# Autodesk Inventor assembly: KickerPCB_Unit
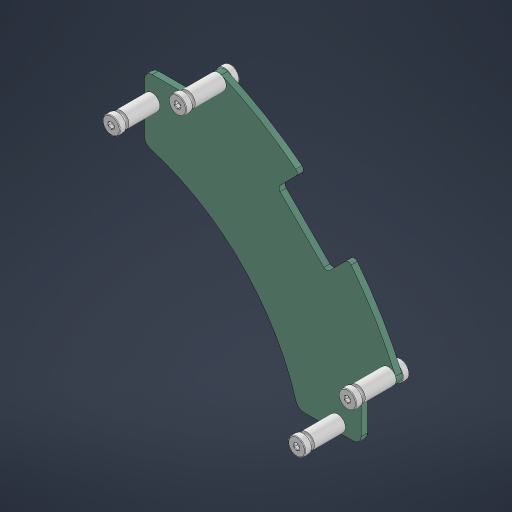
[picture p0: Inventor's stored thumbnail of the model, 512x512]
Saved by Autodesk Inventor 2024.2 (Build 282272000, 272)
## iProperties
Created: 2024-01-10
Part Number: KickerPCB_Unit
Document SubType Name: Assembly
Designer: Hanaoka
Author: Hanaoka
## Documents named in this file (4)
- G:\共有ドライブ\reRo\05_個人\hanaoka\inventor\PCBs\KickerPCB_Unit.iam
- G:\共有ドライブ\reRo\05_個人\hanaoka\inventor\PCBs\MotorDriver_PCB.ipt
- G:\共有ドライブ\reRo\05_個人\hanaoka\inventor\Spacer\Spacer_M2x8.ipt
- G:\共有ドライブ\reRo\05_個人\hanaoka\inventor\Screw\M2x4\M2x4.ipt
## Components (13 placed, 3 different names)
1. MotorDriver_PCB:1 — 挿入:1, 挿入:2, 挿入:3, 挿入:4, 挿入:9, 挿入:10, 挿入:11, 挿入:12
2. Spacer_M2x8:1 — 挿入:4, 挿入:8
3. Spacer_M2x8:2 — 挿入:2, 挿入:6
4. Spacer_M2x8:3 — 挿入:3, 挿入:7
5. Spacer_M2x8:4 — 挿入:1, 挿入:5
6. M2x4:1 — 挿入:5
7. M2x4:2 — 挿入:7
8. M2x4:3 — 挿入:6
9. M2x4:4 — 挿入:8
10. M2x4:5 — 挿入:9
11. M2x4:6 — 挿入:10
12. M2x4:7 — 挿入:11
13. M2x4:8 — 挿入:12
## Relationships (12: Insert 12)
- 挿入:1 [Insert]: MotorDriver_PCB:1 ↔ Spacer_M2x8:4
- 挿入:2 [Insert]: MotorDriver_PCB:1 ↔ Spacer_M2x8:2
- 挿入:3 [Insert]: MotorDriver_PCB:1 ↔ Spacer_M2x8:3
- 挿入:4 [Insert]: MotorDriver_PCB:1 ↔ Spacer_M2x8:1
- 挿入:5 [Insert] (1 mm): Spacer_M2x8:4 ↔ M2x4:1
- 挿入:6 [Insert] (1 mm): Spacer_M2x8:2 ↔ M2x4:3
- 挿入:7 [Insert] (1 mm): Spacer_M2x8:3 ↔ M2x4:2
- 挿入:8 [Insert] (1 mm): Spacer_M2x8:1 ↔ M2x4:4
- 挿入:9 [Insert]: MotorDriver_PCB:1 ↔ M2x4:5
- 挿入:10 [Insert]: MotorDriver_PCB:1 ↔ M2x4:6
- 挿入:11 [Insert]: MotorDriver_PCB:1 ↔ M2x4:7
- 挿入:12 [Insert]: MotorDriver_PCB:1 ↔ M2x4:8
